# Autodesk Inventor assembly: Interrupter
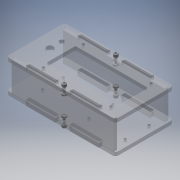
[picture p0: Inventor's stored thumbnail of the model, 180x180]
Saved by Autodesk Inventor 2016 (Build 200138000, 138)
## iProperties
Created: 2018-05-24
Part Number: Interrupter
Document SubType Name: Assembly
Designer: Phil Erle
Author: Phil Erle
## Documents named in this file (6)
- C:\Users\Phil Erle\Desktop\Adrastea\Interrupter.iam
- C:\Users\Phil Erle\Desktop\Adrastea\Interrupter_Bottom.ipt
- C:\Users\Phil Erle\Desktop\Adrastea\Interrupter_Side.ipt
- C:\Users\Phil Erle\Desktop\Adrastea\Interrupter_Top.ipt
- C:\Users\Phil Erle\Desktop\Adrastea\Normteile\Muttern\mutter_din934_m3-6.ipt
- C:\Users\Phil Erle\Desktop\Adrastea\Normteile\Schrauben\M3\din_en_iso_4762_m3x10.ipt
## Components (12 placed, 5 different names)
1. Interrupter_Bottom:1 — Mate:1, Mate:2, Flush:1, Mate:3, Mate:4, Mate:5, Mate:6, Mate:12, Mate:13, Mate:14, Mate:15, Mate:18, Mate:19
2. Interrupter_Side:1 — Mate:1, Mate:5, Mate:9, Mate:10, Mate:11, Mate:13, Mate:29, Mate:30, Mate:32, Mate:33
3. Interrupter_Top:1 — Mate:9, Mate:10, Mate:11, Mate:16, Mate:17, Mate:20, Mate:21
4. Interrupter_Side:2 — Mate:2, Mate:6, Mate:12, Mate:22, Mate:23, Mate:24, Mate:26
5. mutter_din934_m3-6:1 — Mate:31, Mate:32, Mate:33
6. mutter_din934_m3-6:2 — Mate:23, Mate:24, Mate:25
7. mutter_din934_m3-6:3 — Mate:22, Mate:26, Mate:27
8. mutter_din934_m3-6:4 — Mate:28, Mate:29, Mate:30
9. din_en_iso_4762_m3x10:1 — Mate:14, Mate:18, Mate:31
10. din_en_iso_4762_m3x10:2 — Mate:16, Mate:21, Mate:27
11. din_en_iso_4762_m3x10:3 — Mate:17, Mate:20, Mate:28
12. din_en_iso_4762_m3x10:4 — Mate:15, Mate:19, Mate:25
## Relationships (32: Mate 31, Flush 1)
- Mate:1: Interrupter_Bottom:1 ↔ Interrupter_Side:1
- Mate:2: Interrupter_Bottom:1 ↔ Interrupter_Side:2
- Flush:1: Interrupter_Bottom:1
- Mate:3: Interrupter_Bottom:1
- Mate:4: Interrupter_Bottom:1
- Mate:5: Interrupter_Bottom:1 ↔ Interrupter_Side:1
- Mate:6: Interrupter_Bottom:1 ↔ Interrupter_Side:2
- Mate:9: Interrupter_Side:1 ↔ Interrupter_Top:1
- Mate:10: Interrupter_Side:1 ↔ Interrupter_Top:1
- Mate:11: Interrupter_Side:1 ↔ Interrupter_Top:1
- Mate:12: Interrupter_Bottom:1 ↔ Interrupter_Side:2
- Mate:13: Interrupter_Bottom:1 ↔ Interrupter_Side:1
- Mate:14: Interrupter_Bottom:1 ↔ din_en_iso_4762_m3x10:1
- Mate:15: Interrupter_Bottom:1 ↔ din_en_iso_4762_m3x10:4
- Mate:16: Interrupter_Top:1 ↔ din_en_iso_4762_m3x10:2
- Mate:17: Interrupter_Top:1 ↔ din_en_iso_4762_m3x10:3
- Mate:18: Interrupter_Bottom:1 ↔ din_en_iso_4762_m3x10:1
- Mate:19: Interrupter_Bottom:1 ↔ din_en_iso_4762_m3x10:4
- Mate:20: Interrupter_Top:1 ↔ din_en_iso_4762_m3x10:3
- Mate:21: Interrupter_Top:1 ↔ din_en_iso_4762_m3x10:2
- Mate:22: Interrupter_Side:2 ↔ mutter_din934_m3-6:3
- Mate:23: Interrupter_Side:2 ↔ mutter_din934_m3-6:2
- Mate:24: Interrupter_Side:2 ↔ mutter_din934_m3-6:2
- Mate:25: mutter_din934_m3-6:2 ↔ din_en_iso_4762_m3x10:4
- Mate:26: Interrupter_Side:2 ↔ mutter_din934_m3-6:3
- Mate:27: mutter_din934_m3-6:3 ↔ din_en_iso_4762_m3x10:2
- Mate:28: mutter_din934_m3-6:4 ↔ din_en_iso_4762_m3x10:3
- Mate:29: Interrupter_Side:1 ↔ mutter_din934_m3-6:4
- Mate:30: Interrupter_Side:1 ↔ mutter_din934_m3-6:4
- Mate:31: mutter_din934_m3-6:1 ↔ din_en_iso_4762_m3x10:1
- Mate:32: Interrupter_Side:1 ↔ mutter_din934_m3-6:1
- Mate:33: Interrupter_Side:1 ↔ mutter_din934_m3-6:1
